# Autodesk Inventor assembly: Hand and Wrist Assembly
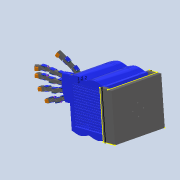
[picture p0: Inventor's stored thumbnail of the model, 180x180]
Saved by Autodesk Inventor 2020 (Build 240168000, 168)
## iProperties
Created: 2020-04-20
Part Number: Hand and Wrist Assembly
Document SubType Name: Assembly
Designer: ttail
Author: ttail
## Documents named in this file (4)
- C:\Users\sami_\Documents\V1.6\Workgroups\NotInProject\Hand and Wrist Assembly.iam
- C:\Users\sami_\Documents\V1.6\Workgroups\NotInProject\Inventor Wrist\Inventor wrist.iam
- C:\Users\sami_\Documents\V1.6\Workgroups\NotInProject\Complete Assembly.iam
- C:\Users\sami_\Documents\V1.6\Workgroups\NotInProject\Inventor Wrist\Mounting Bracket.ipt
## Components (3 placed, 3 different names)
1. Inventor wrist:1 [sub-assembly] — Mate:1, Mate:2, Mate:3, Rigid:1
2. Complete Assembly:1 [sub-assembly] — Mate:1, Mate:2, Mate:3
3. Mounting Bracket:1 — Rigid:1
## Relationships (4: Mate 3, WeldJoint 1)
- Mate:1: Inventor wrist:1 ↔ Complete Assembly:1
- Mate:2: Inventor wrist:1 ↔ Complete Assembly:1
- Mate:3: Inventor wrist:1 ↔ Complete Assembly:1
- Rigid:1 [WeldJoint]: Inventor wrist:1 ↔ Mounting Bracket:1
